# Autodesk Inventor assembly: carrier12
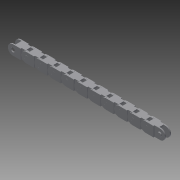
[picture p0: Inventor's stored thumbnail of the model, 180x180]
Saved by Autodesk Inventor 2013 (Build 170138000, 138)
## iProperties
Created: 2013-01-14
Part Number: carrier12
Document SubType Name: Assembly
Designer: Istvan
Author: Istvan
## Documents named in this file (2)
- E:\GitHub\Crown-Fire\CAD\Electronics\carrier\carrier12.iam
- E:\GitHub\Crown-Fire\CAD\Electronics\carrier\carrierSegment.ipt
## Components (11 placed, 1 different names)
1. carrierSegment:1 — Mate:1, Mate:17
2. carrierSegment:2 — Mate:1, Mate:2, Mate:17, Mate:18
3. carrierSegment:3 — Mate:2, Mate:3, Mate:18, Mate:19
4. carrierSegment:4 — Mate:3, Mate:4, Mate:19, Mate:20
5. carrierSegment:5 — Mate:4, Mate:5, Mate:20, Mate:21
6. carrierSegment:6 — Mate:5, Mate:6, Mate:21, Mate:22
7. carrierSegment:7 — Mate:6, Mate:7, Mate:22, Mate:23
8. carrierSegment:8 — Mate:7, Mate:8, Mate:23, Mate:24
9. carrierSegment:9 — Mate:8, Mate:9, Mate:24, Mate:25
10. carrierSegment:10 — Mate:9, Mate:10, Mate:25, Mate:26
11. carrierSegment:11 — Mate:10, Mate:26
## Relationships (20: Mate 20)
- Mate:1: carrierSegment:1 ↔ carrierSegment:2
- Mate:2: carrierSegment:2 ↔ carrierSegment:3
- Mate:3: carrierSegment:3 ↔ carrierSegment:4
- Mate:4: carrierSegment:4 ↔ carrierSegment:5
- Mate:5: carrierSegment:5 ↔ carrierSegment:6
- Mate:6: carrierSegment:6 ↔ carrierSegment:7
- Mate:7: carrierSegment:7 ↔ carrierSegment:8
- Mate:8: carrierSegment:8 ↔ carrierSegment:9
- Mate:9: carrierSegment:9 ↔ carrierSegment:10
- Mate:10: carrierSegment:10 ↔ carrierSegment:11
- Mate:17: carrierSegment:1 ↔ carrierSegment:2
- Mate:18: carrierSegment:2 ↔ carrierSegment:3
- Mate:19: carrierSegment:3 ↔ carrierSegment:4
- Mate:20: carrierSegment:4 ↔ carrierSegment:5
- Mate:21: carrierSegment:5 ↔ carrierSegment:6
- Mate:22: carrierSegment:6 ↔ carrierSegment:7
- Mate:23: carrierSegment:7 ↔ carrierSegment:8
- Mate:24: carrierSegment:8 ↔ carrierSegment:9
- Mate:25: carrierSegment:9 ↔ carrierSegment:10
- Mate:26: carrierSegment:10 ↔ carrierSegment:11
